# Autodesk Inventor assembly: RR-PCSS-2021-3M1-ZŁ
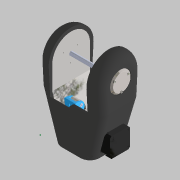
[picture p0: Inventor's stored thumbnail of the model, 180x180]
Saved by Autodesk Inventor 2021 (Build 250183000, 183)
## iProperties
Created: 2021-09-29
Part Number: RR-PCSS-2021-3M1-ZŁ
Document SubType Name: Assembly
Designer: marci
Author: marci
## Documents named in this file (15)
- C:\Users\marci\Desktop\Projekt ramienia\3M1D\RR-PCSS-2021-3M1-ZŁ.iam
- C:\Users\marci\Desktop\Projekt ramienia\3M1D\Część11.ipt
- C:\Users\marci\Desktop\Projekt ramienia\3M1D\RR-PCSS-2021-3M1Db.ipt
- C:\Users\marci\Desktop\Projekt ramienia\3M1D\RR-PCSS-2021-MSK.ipt
- C:\Users\marci\Desktop\Projekt ramienia\3M1D\Nema 17 Reductor.ipt
- C:\Users\marci\Desktop\Projekt ramienia\3M1D\Pulley 8mm IGNIS.ipt
- C:\Users\marci\Desktop\Projekt ramienia\Nowy folder\pl-PL\ISO 4762(2)\ISO 4762 - M3 x 6ISO.ipt
- C:\Users\marci\Desktop\Projekt ramienia\Nowy folder\pl-PL\ANSI B18.3.1M(6)\ANSI B18.3.1M - M3x0,5 x 45(1).ipt
- C:\Users\marci\Desktop\Projekt ramienia\3M1D\T3M1.iam
- C:\Users\marci\Desktop\Projekt ramienia\3M1D\RR-PCSS-2021-3M1Da.ipt
- C:\Users\marci\Desktop\Projekt ramienia\3M1D\8mm Bearing.ipt
- C:\Users\marci\Desktop\Projekt ramienia\3M1D\Smooth bar 8mm x 121mm.ipt
- C:\Users\marci\Desktop\Projekt ramienia\3M1D\Tapa 3M1C.ipt
- C:\Users\marci\Desktop\Projekt ramienia\Nowy folder\pl-PL\ISO 4762(2)\ISO 4762 - M3 x 25ISO.ipt
- C:\Users\marci\Desktop\Projekt ramienia\Nowy folder\pl-PL\ISO 4035(2)\ISO 4035 - M3 - ISO.ipt
## Components (27 placed, 14 different names)
1. Część11:1 — Równoległe:1, Zestawiające:2, Zestawiające:3, Równoległe:2, Zestawiające:4, Zestawiające:16, Wstawiające:3
2. RR-PCSS-2021-3M1Db:1 — Równoległe:1, Zestawiające:2, Zestawiające:16, Zestawiające:17, Równoległe:3, Wstawiające:4, Wstawiające:7, Zestawiające:35, Zestawiające:37
3. RR-PCSS-2021-MSK:1 — Zestawiające:3, Równoległe:2, Zestawiające:4, Wstawiające:1, Zestawiające:5, Zestawiające:6, Zestawiające:7, Zestawiające:8, Zestawiające:9, Zestawiające:10, Zestawiające:11, Zestawiające:12, Zestawiające:13, Zestawiające:14
4. Nema 17 Reductor:1 — Wstawiające:1, Wstawiające:2
5. Pulley 8mm IGNIS:1 — Wstawiające:2
6. ISO 4762 M3 x 6:1 — Zestawiające:5, Zestawiające:6
7. ISO 4762 M3 x 6:2 — Zestawiające:7, Zestawiające:8
8. ISO 4762 M3 x 6:3 — Zestawiające:9, Zestawiające:10
9. ISO 4762 M3 x 6:4 — Zestawiające:11, Zestawiające:12
10. Wkręt z łbem o zmniejszonych wymiarach z gniazdem kutym - Metryczny M3x0,5 x 45:1 — Zestawiające:13, Zestawiające:14, Zestawiające:15
11. T3M1:1 [sub-assembly] — Zestawiające:15
12. RR-PCSS-2021-3M1Da:1 — Zestawiające:17, Równoległe:3, Wstawiające:3, Wstawiające:5, Wstawiające:8, Zestawiające:30, Zestawiające:31, Zestawiające:32, Zestawiające:33, Zestawiające:34, Zestawiające:36
13. 8mm Bearing:1 — Wstawiające:5
14. 8mm Bearing:2 — Wstawiające:4, Wstawiające:9
15. Smooth bar 8mm x 121mm:1 — Wstawiające:9
16. Tapa 3M1C:1 — Wstawiające:8, Zestawiające:24, Zestawiające:25, Zestawiające:26, Zestawiające:27, Zestawiające:28, Zestawiające:29
17. Tapa 3M1C:2 — Wstawiające:7, Zestawiające:18, Zestawiające:19, Zestawiające:20, Zestawiające:21, Zestawiające:22, Zestawiające:23
18. ISO 4762 M3 x 25:1 — Zestawiające:18, Zestawiające:19
19. ISO 4762 M3 x 25:2 — Zestawiające:20, Zestawiające:21
20. ISO 4762 M3 x 25:3 — Zestawiające:22, Zestawiające:23
21. ISO 4762 M3 x 25:4 — Zestawiające:24, Zestawiające:25
22. ISO 4762 M3 x 25:5 — Zestawiające:26, Zestawiające:27
23. ISO 4762 M3 x 25:6 — Zestawiające:28, Zestawiające:29
24. Wkręt z łbem o zmniejszonych wymiarach z gniazdem kutym - Metryczny M3x0,5 x 45:2 — Zestawiające:30, Zestawiające:31
25. ISO 4035 M3:1 — Zestawiające:34, Zestawiające:35
26. Wkręt z łbem o zmniejszonych wymiarach z gniazdem kutym - Metryczny M3x0,5 x 45:3 — Zestawiające:32, Zestawiające:33
27. ISO 4035 M3:2 — Zestawiające:36, Zestawiające:37
## Relationships (47: Mate 36, Insert 8, Flush 3)
- Równoległe:1 [Flush]: Część11:1 ↔ RR-PCSS-2021-3M1Db:1
- Zestawiające:2 [Mate]: Część11:1 ↔ RR-PCSS-2021-3M1Db:1
- Zestawiające:3 [Mate]: Część11:1 ↔ RR-PCSS-2021-MSK:1
- Równoległe:2 [Flush] (-45.724 mm): Część11:1 ↔ RR-PCSS-2021-MSK:1
- Zestawiające:4 [Mate] (22 mm): Część11:1 ↔ RR-PCSS-2021-MSK:1
- Wstawiające:1 [Insert]: RR-PCSS-2021-MSK:1 ↔ Nema 17 Reductor:1
- Wstawiające:2 [Insert]: Nema 17 Reductor:1 ↔ Pulley 8mm IGNIS:1
- Zestawiające:5 [Mate]: RR-PCSS-2021-MSK:1 ↔ ISO 4762 M3 x 6:1
- Zestawiające:6 [Mate]: RR-PCSS-2021-MSK:1 ↔ ISO 4762 M3 x 6:1
- Zestawiające:7 [Mate]: RR-PCSS-2021-MSK:1 ↔ ISO 4762 M3 x 6:2
- Zestawiające:8 [Mate]: RR-PCSS-2021-MSK:1 ↔ ISO 4762 M3 x 6:2
- Zestawiające:9 [Mate]: RR-PCSS-2021-MSK:1 ↔ ISO 4762 M3 x 6:3
- Zestawiające:10 [Mate]: RR-PCSS-2021-MSK:1 ↔ ISO 4762 M3 x 6:3
- Zestawiające:11 [Mate]: RR-PCSS-2021-MSK:1 ↔ ISO 4762 M3 x 6:4
- Zestawiające:12 [Mate]: RR-PCSS-2021-MSK:1 ↔ ISO 4762 M3 x 6:4
- Zestawiające:13 [Mate]: RR-PCSS-2021-MSK:1 ↔ Wkręt z łbem o zmniejszonych wymiarach z gniazdem kutym - Metryczny M3x0,5 x 45:1
- Zestawiające:14 [Mate]: RR-PCSS-2021-MSK:1 ↔ Wkręt z łbem o zmniejszonych wymiarach z gniazdem kutym - Metryczny M3x0,5 x 45:1
- Zestawiające:15 [Mate]: Wkręt z łbem o zmniejszonych wymiarach z gniazdem kutym - Metryczny M3x0,5 x 45:1 ↔ T3M1:1
- Zestawiające:16 [Mate]: Część11:1 ↔ RR-PCSS-2021-3M1Db:1
- Zestawiające:17 [Mate]: RR-PCSS-2021-3M1Db:1 ↔ RR-PCSS-2021-3M1Da:1
- Równoległe:3 [Flush]: RR-PCSS-2021-3M1Db:1 ↔ RR-PCSS-2021-3M1Da:1
- Wstawiające:3 [Insert]: Część11:1 ↔ RR-PCSS-2021-3M1Da:1
- Wstawiające:4 [Insert]: RR-PCSS-2021-3M1Db:1 ↔ 8mm Bearing:2
- Wstawiające:5 [Insert]: RR-PCSS-2021-3M1Da:1 ↔ 8mm Bearing:1
- Wstawiające:7 [Insert]: RR-PCSS-2021-3M1Db:1 ↔ Tapa 3M1C:2
- Wstawiające:8 [Insert]: RR-PCSS-2021-3M1Da:1 ↔ Tapa 3M1C:1
- Wstawiające:9 [Insert]: 8mm Bearing:2 ↔ Smooth bar 8mm x 121mm:1
- Zestawiające:18 [Mate]: Tapa 3M1C:2 ↔ ISO 4762 M3 x 25:1
- Zestawiające:19 [Mate]: Tapa 3M1C:2 ↔ ISO 4762 M3 x 25:1
- Zestawiające:20 [Mate]: Tapa 3M1C:2 ↔ ISO 4762 M3 x 25:2
- Zestawiające:21 [Mate]: Tapa 3M1C:2 ↔ ISO 4762 M3 x 25:2
- Zestawiające:22 [Mate]: Tapa 3M1C:2 ↔ ISO 4762 M3 x 25:3
- Zestawiające:23 [Mate]: Tapa 3M1C:2 ↔ ISO 4762 M3 x 25:3
- Zestawiające:24 [Mate]: Tapa 3M1C:1 ↔ ISO 4762 M3 x 25:4
- Zestawiające:25 [Mate]: Tapa 3M1C:1 ↔ ISO 4762 M3 x 25:4
- Zestawiające:26 [Mate]: Tapa 3M1C:1 ↔ ISO 4762 M3 x 25:5
- Zestawiające:27 [Mate]: Tapa 3M1C:1 ↔ ISO 4762 M3 x 25:5
- Zestawiające:28 [Mate]: Tapa 3M1C:1 ↔ ISO 4762 M3 x 25:6
- Zestawiające:29 [Mate]: Tapa 3M1C:1 ↔ ISO 4762 M3 x 25:6
- Zestawiające:30 [Mate]: RR-PCSS-2021-3M1Da:1 ↔ Wkręt z łbem o zmniejszonych wymiarach z gniazdem kutym - Metryczny M3x0,5 x 45:2
- Zestawiające:31 [Mate]: RR-PCSS-2021-3M1Da:1 ↔ Wkręt z łbem o zmniejszonych wymiarach z gniazdem kutym - Metryczny M3x0,5 x 45:2
- Zestawiające:32 [Mate]: RR-PCSS-2021-3M1Da:1 ↔ Wkręt z łbem o zmniejszonych wymiarach z gniazdem kutym - Metryczny M3x0,5 x 45:3
- Zestawiające:33 [Mate]: RR-PCSS-2021-3M1Da:1 ↔ Wkręt z łbem o zmniejszonych wymiarach z gniazdem kutym - Metryczny M3x0,5 x 45:3
- Zestawiające:34 [Mate]: RR-PCSS-2021-3M1Da:1 ↔ ISO 4035 M3:1
- Zestawiające:35 [Mate]: RR-PCSS-2021-3M1Db:1 ↔ ISO 4035 M3:1
- Zestawiające:36 [Mate]: RR-PCSS-2021-3M1Da:1 ↔ ISO 4035 M3:2
- Zestawiające:37 [Mate]: RR-PCSS-2021-3M1Db:1 ↔ ISO 4035 M3:2
